# Autodesk Inventor assembly: Wing Left
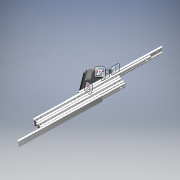
[picture p0: Inventor's stored thumbnail of the model, 180x180]
Saved by Autodesk Inventor 2019 (Build 230136000, 136)
## iProperties
Part Number: Wing Left
Document SubType Name: Assembly
Designer: Delta
Author: Delta
## Documents named in this file (5)
- C:\Robotics\CAD\2019-20_CAD\Collection\Wing Left.iam
- C:\Robotics\CAD\2019-20_CAD\Collection\Triangle axle slide connector.ipt
- C:\Robotics\CAD\COTSParts\Rev\REV-41-1683 Bear Blocks.ipt
- C:\Robotics\CAD\COTSParts\Misumi_Slides\AIS2018\SAR330.iam
- C:\Robotics\CAD\2018-19_CAD\2019-20_CAD\offseason\slide conector.ipt
## Components (7 placed, 4 different names)
1. Triangle axle slide connector:1 — Mate:3, Mate:4, Angle:1, Mate:13, Mate:27, Mate:28
2. REV-41-1683 Bear Blocks:1 — Mate:3, Mate:4, Angle:1
3. SAR330:1 [sub-assembly] — Mate:13, Mate:15, Mate:16, Mate:17, Mate:27, Mate:28
4. SAR330:2 [sub-assembly] — Mate:24, Mate:25, Mate:26
5. SAR330:3 [sub-assembly] — Mate:18, Mate:19, Mate:20, Mate:21, Mate:22, Mate:23
6. slide conector:1 — Mate:15, Mate:16, Mate:17, Mate:18, Mate:19, Mate:20
7. slide conector:2 — Mate:21, Mate:22, Mate:23, Mate:24, Mate:25, Mate:26
## Relationships (18: Mate 17, Angle 1)
- Mate:3: Triangle axle slide connector:1 ↔ REV-41-1683 Bear Blocks:1
- Mate:4: Triangle axle slide connector:1 ↔ REV-41-1683 Bear Blocks:1
- Angle:1 (0 deg): Triangle axle slide connector:1 ↔ REV-41-1683 Bear Blocks:1
- Mate:13: Triangle axle slide connector:1 ↔ SAR330:1
- Mate:15: SAR330:1 ↔ slide conector:1
- Mate:16: SAR330:1 ↔ slide conector:1
- Mate:17: SAR330:1 ↔ slide conector:1
- Mate:18: SAR330:3 ↔ slide conector:1
- Mate:19: SAR330:3 ↔ slide conector:1
- Mate:20: SAR330:3 ↔ slide conector:1
- Mate:21: SAR330:3 ↔ slide conector:2
- Mate:22: SAR330:3 ↔ slide conector:2
- Mate:23: SAR330:3 ↔ slide conector:2
- Mate:24: SAR330:2 ↔ slide conector:2
- Mate:25: SAR330:2 ↔ slide conector:2
- Mate:26: SAR330:2 ↔ slide conector:2
- Mate:27: Triangle axle slide connector:1 ↔ SAR330:1
- Mate:28: Triangle axle slide connector:1 ↔ SAR330:1
